# Autodesk Inventor assembly: TapaSeguridad
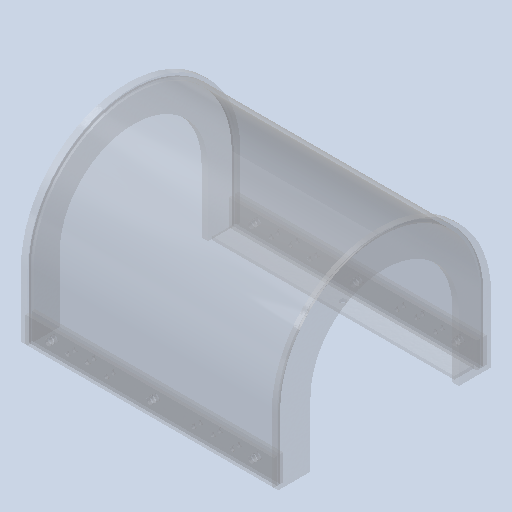
[picture p0: Inventor's stored thumbnail of the model, 512x512]
Saved by Autodesk Inventor 2022 (Build 260153000, 153)
## iProperties
Created: 2018-06-05
Part Number: TapaSeguridad
Material: Genérico
Document SubType Name: Assembly
Designer: Cristiano
Author: Cristiano
## Documents named in this file (5)
- G:\Mi unidad\UTEC\Proyectos\Flor de Lana\Diseño 20191119\TapaSeguridad\TapaSeguridad.iam
- G:\Mi unidad\UTEC\Proyectos\Flor de Lana\Diseño 20191119\TapaSeguridad\Sup.Acrilico.ipt
- G:\Mi unidad\UTEC\Proyectos\Flor de Lana\Diseño 20191119\TapaSeguridad\Acrilico.ipt
- G:\Mi unidad\UTEC\Proyectos\Flor de Lana\Diseño 20191119\TapaSeguridad\Base.pin.Seg.ipt
- G:\Mi unidad\UTEC\Proyectos\Flor de Lana\Diseño 20191119\TapaSeguridad\Tapa Frontar y Posterior.ipt
## Components (8 placed, 4 different names)
1. Sup.Acrilico:1 — Rígido:12
2. Sup.Acrilico:2 — Rígido:4, Rígido:11
3. Sup.Acrilico:3 — Rígido:7
4. Sup.Acrilico:4 — Rígido:8
5. Acrilico:1 — Rígido:12, Rígido:4, Rígido:7, Rígido:8, Nivelación:1, Nivelación:2, Nivelación:3, Rigid:13, Rigid:14
6. Base.pin.Seg:1 — Rígido:11
7. Tapa Frontar y Posterior:1 — Rigid:14
8. Tapa Frontar y Posterior:2 — Rigid:13
## Relationships (10: WeldJoint 7, Flush 3)
- Rígido:12 [WeldJoint]: Sup.Acrilico:1 ↔ Acrilico:1
- Rígido:4 [WeldJoint]: Sup.Acrilico:2 ↔ Acrilico:1
- Rígido:7 [WeldJoint]: Sup.Acrilico:3 ↔ Acrilico:1
- Rígido:8 [WeldJoint]: Sup.Acrilico:4 ↔ Acrilico:1
- Rígido:11 [WeldJoint]: Sup.Acrilico:2 ↔ Base.pin.Seg:1
- Nivelación:1 [Flush]: Acrilico:1
- Nivelación:2 [Flush]: Acrilico:1
- Nivelación:3 [Flush]: Acrilico:1
- Rigid:13 [WeldJoint]: Acrilico:1 ↔ Tapa Frontar y Posterior:2
- Rigid:14 [WeldJoint]: Acrilico:1 ↔ Tapa Frontar y Posterior:1
